# Autodesk Inventor assembly: scraper
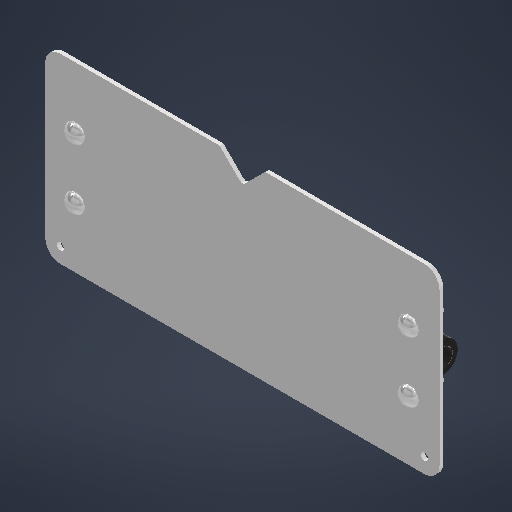
[picture p0: Inventor's stored thumbnail of the model, 512x512]
Saved by Autodesk Inventor 2026.1 (Build 301233000, 233)
## iProperties
Created: 2026-01-07
Part Number: scraper
Document SubType Name: Assembly
Designer: roejo
Author: roejo
## Documents named in this file (5)
- C:\Users\roejo\OneDrive\Documents\7700RKalahariCAD\Robots\Kalahari\Subassemblies\scraper.iam
- C:\Users\roejo\OneDrive\Documents\7700RKalahariCAD\Robots\Kalahari\Poly\matchloader.ipt
- C:\Users\roejo\OneDrive\Documents\7700RKalahariCAD\Library\VEX-CAD-Inventor-1.4.2\Motion\Shaft HS\HS Pillow Bearing Block.ipt
- C:\Users\roejo\OneDrive\Documents\7700RKalahariCAD\Library\VEX-CAD-Inventor-1.4.2\Structure\Hardware\Screw Aluminum - Flat Head\AScrew Flat Head Threaded .500.ipt
- C:\Users\roejo\OneDrive\Documents\7700RKalahariCAD\Library\VEX-CAD-Inventor-1.4.2\Structure\Hardware\alu_nylock.ipt
## Components (11 placed, 4 different names)
1. matchloader:1 — Insert:1, Insert:2, Insert:3, Insert:4, Insert:5, Insert:6, Insert:7, Insert:8
2. HS Pillow Bearing Block:1 — Insert:3, Insert:4, Insert:11, Insert:12
3. HS Pillow Bearing Block:2 — Insert:1, Insert:2, Insert:9, Insert:10
4. AScrew Flat Head Threaded .500:1 — Insert:6
5. AScrew Flat Head Threaded .500:2 — Insert:7
6. AScrew Flat Head Threaded .500:3 — Insert:5
7. AScrew Flat Head Threaded .500:4 — Insert:8
8. alu_nylock:1 — Insert:9
9. alu_nylock:2 — Insert:11
10. alu_nylock:3 — Insert:10
11. alu_nylock:4 — Insert:12
## Relationships (12: Insert 12)
- Insert:1: matchloader:1 ↔ HS Pillow Bearing Block:2
- Insert:2: matchloader:1 ↔ HS Pillow Bearing Block:2
- Insert:3: matchloader:1 ↔ HS Pillow Bearing Block:1
- Insert:4: matchloader:1 ↔ HS Pillow Bearing Block:1
- Insert:5: matchloader:1 ↔ AScrew Flat Head Threaded .500:3
- Insert:6: matchloader:1 ↔ AScrew Flat Head Threaded .500:1
- Insert:7: matchloader:1 ↔ AScrew Flat Head Threaded .500:2
- Insert:8: matchloader:1 ↔ AScrew Flat Head Threaded .500:4
- Insert:9: HS Pillow Bearing Block:2 ↔ alu_nylock:1
- Insert:10: HS Pillow Bearing Block:2 ↔ alu_nylock:3
- Insert:11: HS Pillow Bearing Block:1 ↔ alu_nylock:2
- Insert:12: HS Pillow Bearing Block:1 ↔ alu_nylock:4
